# Autodesk Inventor assembly: Foot_MIR
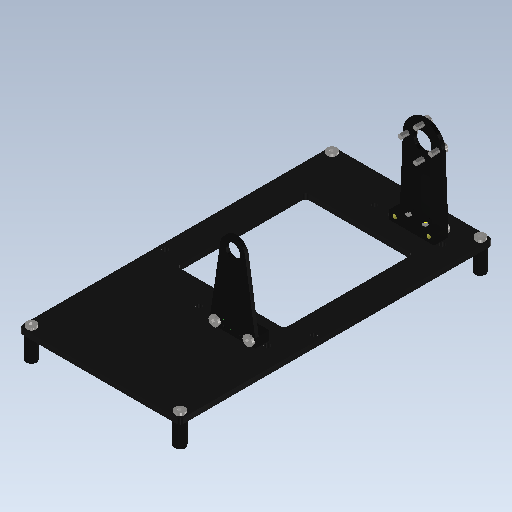
[picture p0: Inventor's stored thumbnail of the model, 512x512]
Saved by Autodesk Inventor 2020.4 (Build 244396000, 396)
## iProperties
Created: 2022-06-03
Part Number: Foot_MIR
Document SubType Name: Assembly
Designer: Masato Kubotera
Author: Masato Kubotera
## Documents named in this file (10)
- C:\Users\Masato\Desktop\SUSTAINA-OP\LowerBody\Foot\Foot_MIR.iam
- C:\Users\Masato\Desktop\SUSTAINA-OP\LowerBody\Foot\Sole_frame.ipt
- C:\Users\Masato\Desktop\SUSTAINA-OP\LowerBody\Foot\Foot_front_frame.ipt
- C:\Users\Masato\Desktop\SUSTAINA-OP\LowerBody\Foot\Foot_back_frame.ipt
- C:\Users\Masato\Desktop\SUSTAINA-OP\LowerBody\Foot\Foot_root_block.ipt
- C:\Users\Masato\Desktop\SUSTAINA-OP\ReadyMade\Spacer\ASL-313BE.ipt
- C:\Users\Masato\Desktop\SUSTAINA-OP\ReadyMade\Screw\M3-10.ipt
- C:\Users\Masato\Desktop\SUSTAINA-OP\ReadyMade\Screw\M3-6.ipt
- C:\Users\Masato\Desktop\SUSTAINA-OP\ReadyMade\Screw\M3-8.ipt
- C:\Users\Masato\Desktop\SUSTAINA-OP\ReadyMade\Screw\M2_6-6.ipt
## Components (25 placed, 9 different names)
1. Sole_frame:1 — 挿入:2, 挿入:1, 挿入:4, 挿入:3, 挿入:13, 挿入:14, 挿入:15, 挿入:16, 挿入:21, 角度:4, 挿入:22, 挿入:23, 挿入:24, 挿入:25, 挿入:26, 挿入:27, 挿入:28
2. Foot_front_frame:1 — メイト:2, メイト:1, 挿入:6, 挿入:5, 挿入:9, 挿入:10
3. Foot_back_frame:1 — 挿入:8, 挿入:7, 挿入:11, 挿入:12, 挿入:17, 挿入:18, 挿入:19, 挿入:20
4. Foot_root_block:1 — 挿入:6, 挿入:5, 挿入:2, 挿入:1
5. Foot_root_block:2 — 挿入:8, 挿入:7, 挿入:4, 挿入:3
6. ASL-313BE:1 — メイト:3, 挿入:21, 角度:4, 角度:1, 角度:2, 角度:3
7. ASL-313BE:2 — 挿入:22, 角度:1
8. ASL-313BE:3 — 挿入:23, 角度:2
9. ASL-313BE:4 — 挿入:24, 角度:3
10. M3-10:1 — 挿入:25
11. M3-10:2 — 挿入:26
12. M3-10:3 — 挿入:27
13. M3-10:4 — 挿入:28
14. M3-6:1 — 挿入:9
15. M3-6:2 — 挿入:10
16. M3-6:3 — 挿入:11
17. M3-6:4 — 挿入:12
18. M3-8:1 — 挿入:13
19. M3-8:2 — 挿入:14
20. M3-8:3 — 挿入:15
21. M3-8:4 — 挿入:16
22. M2_6-6:1 — 挿入:17
23. M2_6-6:2 — 挿入:18
24. M2_6-6:3 — 挿入:19
25. M2_6-6:4 — 挿入:20
## Relationships (35: Insert 28, Angle 4, Mate 3)
- メイト:2 [Mate]: Foot_front_frame:1
- メイト:1 [Mate]: Foot_front_frame:1
- 挿入:6 [Insert]: Foot_front_frame:1 ↔ Foot_root_block:1
- 挿入:5 [Insert]: Foot_front_frame:1 ↔ Foot_root_block:1
- 挿入:2 [Insert]: Sole_frame:1 ↔ Foot_root_block:1
- 挿入:1 [Insert]: Sole_frame:1 ↔ Foot_root_block:1
- 挿入:8 [Insert]: Foot_back_frame:1 ↔ Foot_root_block:2
- 挿入:7 [Insert]: Foot_back_frame:1 ↔ Foot_root_block:2
- 挿入:4 [Insert]: Sole_frame:1 ↔ Foot_root_block:2
- 挿入:3 [Insert]: Sole_frame:1 ↔ Foot_root_block:2
- 挿入:9 [Insert]: Foot_front_frame:1 ↔ M3-6:1
- 挿入:10 [Insert]: Foot_front_frame:1 ↔ M3-6:2
- 挿入:11 [Insert]: Foot_back_frame:1 ↔ M3-6:3
- 挿入:12 [Insert]: Foot_back_frame:1 ↔ M3-6:4
- 挿入:13 [Insert]: Sole_frame:1 ↔ M3-8:1
- 挿入:14 [Insert]: Sole_frame:1 ↔ M3-8:2
- 挿入:15 [Insert]: Sole_frame:1 ↔ M3-8:3
- 挿入:16 [Insert]: Sole_frame:1 ↔ M3-8:4
- 挿入:17 [Insert]: Foot_back_frame:1 ↔ M2_6-6:1
- 挿入:18 [Insert]: Foot_back_frame:1 ↔ M2_6-6:2
- 挿入:19 [Insert]: Foot_back_frame:1 ↔ M2_6-6:3
- 挿入:20 [Insert]: Foot_back_frame:1 ↔ M2_6-6:4
- メイト:3 [Mate]: ASL-313BE:1
- 挿入:21 [Insert]: Sole_frame:1 ↔ ASL-313BE:1
- 角度:4 [Angle] (0 deg): Sole_frame:1 ↔ ASL-313BE:1
- 挿入:22 [Insert]: Sole_frame:1 ↔ ASL-313BE:2
- 角度:1 [Angle] (0 deg): ASL-313BE:1 ↔ ASL-313BE:2
- 挿入:23 [Insert]: Sole_frame:1 ↔ ASL-313BE:3
- 角度:2 [Angle] (0 deg): ASL-313BE:1 ↔ ASL-313BE:3
- 挿入:24 [Insert]: Sole_frame:1 ↔ ASL-313BE:4
- 角度:3 [Angle] (0 deg): ASL-313BE:1 ↔ ASL-313BE:4
- 挿入:25 [Insert]: Sole_frame:1 ↔ M3-10:1
- 挿入:26 [Insert]: Sole_frame:1 ↔ M3-10:2
- 挿入:27 [Insert]: Sole_frame:1 ↔ M3-10:3
- 挿入:28 [Insert]: Sole_frame:1 ↔ M3-10:4
